# Autodesk Inventor assembly: Manfrotto_501_PL_assem_01
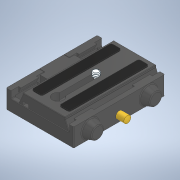
[picture p0: Inventor's stored thumbnail of the model, 180x180]
Saved by Autodesk Inventor 2020 (Build 240168000, 168)
## iProperties
Created: 2015-09-30
Part Number: Manfrotto_501_PL_assem_01
Document SubType Name: Assembly
Designer: Hesekiel
Sending System: SolidWorks 2014
Last Author: istvan1188
Last Saved: 2015-09-30
Author: Hesekiel
## Documents named in this file (4)
- C:\Users\Hesekiel\Desktop\Equatorial-Mount-MUM\Mechanika\Mechanizm elewacji Filip\CAD\manfrotto-quick-release-plate\Manfrotto_501_PL_assem_01.iam
- C:\Users\Hesekiel\Desktop\Equatorial-Mount-MUM\Mechanika\Mechanizm elewacji Filip\CAD\manfrotto-quick-release-plate\manfrotto_501_PL.ipt
- C:\Users\Hesekiel\Desktop\Equatorial-Mount-MUM\Mechanika\Mechanizm elewacji Filip\CAD\manfrotto-quick-release-plate\manfrotto_PL-577_main.ipt
- C:\Users\Hesekiel\Desktop\Equatorial-Mount-MUM\Mechanika\Mechanizm elewacji Filip\CAD\manfrotto-quick-release-plate\1_4_withwort_manfrotto_screw.ipt
## Components (3 placed, 3 different names)
1. manfrotto_501_PL:1 — Mate:1, Flush:1, Mate:2, Mate:3, Mate:4
2. manfrotto_PL-577_main:1 — Mate:1, Flush:1, Mate:2
3. 1_4_withwort_manfrotto_screw:1 — Mate:3, Mate:4
## Relationships (5: Mate 4, Flush 1)
- Mate:1: manfrotto_501_PL:1 ↔ manfrotto_PL-577_main:1
- Flush:1: manfrotto_501_PL:1 ↔ manfrotto_PL-577_main:1
- Mate:2: manfrotto_501_PL:1 ↔ manfrotto_PL-577_main:1
- Mate:3: manfrotto_501_PL:1 ↔ 1_4_withwort_manfrotto_screw:1
- Mate:4: manfrotto_501_PL:1 ↔ 1_4_withwort_manfrotto_screw:1
